# Autodesk Inventor assembly: side of drivetrain
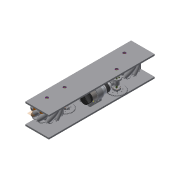
[picture p0: Inventor's stored thumbnail of the model, 180x180]
Saved by Autodesk Inventor 2020 (Build 240168000, 168)
## iProperties
Created: 2019-10-04
Part Number: side of drivetrain
Document SubType Name: Assembly
Designer: ball
Author: ball
## Documents named in this file (7)
- C:\FTC\FTC8863CAD\2019 Robot\Mecanum Drive Train\side of drivetrain.iam
- C:\FTC\FTC8863CAD\2019 Robot\Mecanum Drive Train\wheel with drive motor top.iam
- C:\FTC\FTC8863CAD\2019 Robot\Mecanum Drive Train\wheel with drive motor floor.iam
- C:\FTC\FTC8863CAD\2019 Robot\Mecanum Drive Train\inside wall.ipt
- C:\FTC\FTC8863CAD\2019 Robot\Mecanum Drive Train\center motor mount.ipt
- C:\FTC\FTC8863CAD\2019 Robot\Mecanum Drive Train\outside wall.ipt
- C:\FTC\FTC8863CAD\2019 Robot\Mecanum Drive Train\motor mount cap.ipt
## Components (7 placed, 6 different names)
1. wheel with drive motor top:1 [sub-assembly] — Flush:4, Mate:5, Flush:6, Mate:7, Mate:8, Mate:12, Mate:14
2. wheel with drive motor floor:1 [sub-assembly] — Flush:4, Mate:5, Flush:6, Mate:9, Mate:13
3. inside wall — Mate:7, Mate:8, Mate:9, Mate:11
4. center motor mount:1 — Mate:15, Flush:7, Mate:16, Flush:8, Mate:17, Mate:18
5. outside wall:1 — Mate:12, Mate:13, Mate:14
6. motor mount cap:1 — Mate:15, Flush:7, Mate:18
7. motor mount cap:2 — Mate:16, Flush:8, Mate:17
## Relationships (16: Mate 12, Flush 4)
- Flush:4: wheel with drive motor top:1 ↔ wheel with drive motor floor:1
- Mate:5 (44.3484 mm): wheel with drive motor top:1 ↔ wheel with drive motor floor:1
- Flush:6 (330.2 mm): wheel with drive motor top:1 ↔ wheel with drive motor floor:1
- Mate:7: wheel with drive motor top:1 ↔ inside wall
- Mate:8: wheel with drive motor top:1 ↔ inside wall
- Mate:9: wheel with drive motor floor:1 ↔ inside wall
- Mate:11: inside wall
- Mate:12: wheel with drive motor top:1 ↔ outside wall:1
- Mate:13: wheel with drive motor floor:1 ↔ outside wall:1
- Mate:14: wheel with drive motor top:1 ↔ outside wall:1
- Mate:15 (0.635 mm): center motor mount:1 ↔ motor mount cap:1
- Flush:7: center motor mount:1 ↔ motor mount cap:1
- Mate:16 (0.635 mm): center motor mount:1 ↔ motor mount cap:2
- Flush:8: center motor mount:1 ↔ motor mount cap:2
- Mate:17: center motor mount:1 ↔ motor mount cap:2
- Mate:18: center motor mount:1 ↔ motor mount cap:1
